# Autodesk Inventor assembly: 8inDriveWheel
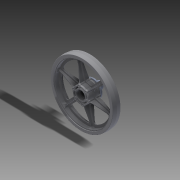
[picture p0: Inventor's stored thumbnail of the model, 180x180]
Saved by Autodesk Inventor 2015 (Build 190159000, 159)
## iProperties
Created: 2015-01-30
Part Number: 8inDriveWheel
Document SubType Name: Assembly
Designer: Kingbob26
Author: Kingbob26
## Documents named in this file (4)
- C:\Users\Kingbob26\Documents\GitHub\2015CAD\actualWheelBase\Drive Base\Parts\8inDriveWheel.iam
- C:\Users\Kingbob26\Documents\GitHub\2015CAD\actualWheelBase\Drive Base\Parts\am0420_8inHub.ipt
- C:\Users\Kingbob26\Documents\GitHub\2015CAD\actualWheelBase\Drive Base\Parts\am0420_8inTread.ipt
- C:\Users\Kingbob26\Documents\GitHub\2015CAD\actualWheelBase\Drive Base\Parts\wheelMount.ipt
## Components (3 placed, 3 different names)
1. am0420_8inHub:1
2. am0420_8inTread:1
3. wheelMount:1
## Relationships (4: Mate 3, Insert 1)
- [Insert]: am0420_8inHub:1 ↔ am0420_8inTread:1
- [Mate]: am0420_8inHub:1 ↔ wheelMount:1
- [Mate]: am0420_8inHub:1 ↔ wheelMount:1
- [Mate]: am0420_8inHub:1 ↔ wheelMount:1
